# Autodesk Inventor assembly: RingL3
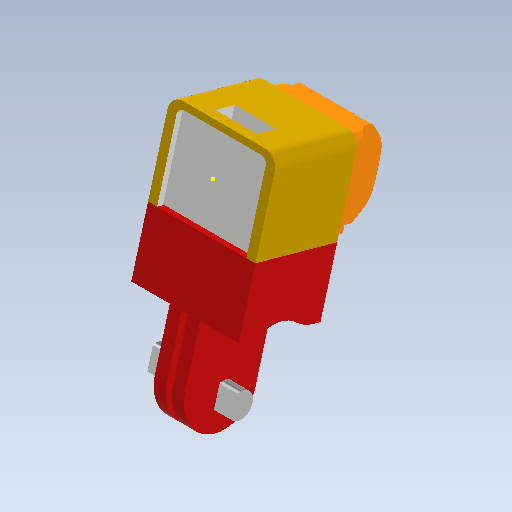
[picture p0: Inventor's stored thumbnail of the model, 512x512]
Saved by Autodesk Inventor 2020 (Build 240168000, 168)
## iProperties
Created: 2020-04-30
Part Number: RingL3
Document SubType Name: Assembly
Designer: sami_
Author: sami_
## Documents named in this file (4)
- C:\Users\sami_\Documents\V1.6\RingL3.iam
- C:\Users\sami_\Documents\V1.6\Workgroups\NotInProject\RING\Fingertip assembly final.iam
- C:\Users\sami_\Documents\V1.6\Workgroups\NotInProject\SHAFT.ipt
- C:\Users\sami_\Documents\V1.6\Workgroups\NotInProject\Fingertiptest2-Solid 2mm base.ipt
## Components (3 placed, 3 different names)
1. Fingertip assembly final:1 [sub-assembly] — Rigid:2
2. SHAFT:1
3. Fingertiptest2-Solid 2mm base:1 — Rigid:2
## Relationships (2: WeldJoint 2)
- [WeldJoint] (3 mm): Fingertip assembly final:1 ↔ SHAFT:1
- Rigid:2 [WeldJoint] (-1 mm): Fingertip assembly final:1 ↔ Fingertiptest2-Solid 2mm base:1
